# Autodesk Inventor assembly: Assembly1
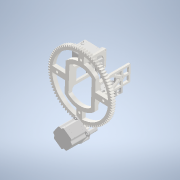
[picture p0: Inventor's stored thumbnail of the model, 180x180]
Saved by Autodesk Inventor 2020 (Build 240168000, 168)
## iProperties
Created: 2019-04-12
Part Number: Assembly1
Document SubType Name: Assembly
Designer: Connor
Author: Connor
## Documents named in this file (7)
- C:\Users\Connor\Desktop\Sentinel CAD\MainAssembly.iam
- C:\Users\Connor\Desktop\Sentinel CAD\MainAssembly\Design Accelerator\GearAssembly.iam
- C:\Users\Connor\Desktop\Sentinel CAD\HoseMount.ipt
- C:\Users\Connor\Desktop\Sentinel CAD\PK266M-01A.ipt
- C:\Users\Connor\Desktop\Sentinel CAD\TopMotorMount.ipt
- C:\Users\Connor\Desktop\Sentinel CAD\NozzleAdapter.ipt
- C:\Users\Connor\Desktop\Sentinel CAD\CameraFilterPlate.ipt
## Components (7 placed, 6 different names)
1. Spur Gears:1 [sub-assembly] — Mate:1, Mate:3, Mate:4, Flush:1, Mate:7
2. PK266M-01A:1 — Mate:1, Mate:3, Mate:4, Mate:5, Mate:6, Angle:1
3. HoseMount:1 — Mate:5, Mate:6, Angle:1, Mate:11, Mate:12, Mate:13, Mate:14, Mate:15, Mate:16
4. TopMotorMount:1 — Flush:1, Mate:7, Mate:8, Mate:9, Mate:10
5. PK266M-01A:2 — Mate:8, Mate:9, Mate:10
6. NozzleAdapter:1 — Mate:11, Mate:12, Mate:13
7. CameraFilterPlate:1 — Mate:14, Mate:15, Mate:16
## Relationships (17: Mate 15, Angle 1, Flush 1)
- Mate:1: Spur Gears:1 ↔ PK266M-01A:1
- Mate:3: Spur Gears:1 ↔ PK266M-01A:1
- Mate:4: Spur Gears:1 ↔ PK266M-01A:1
- Mate:5: PK266M-01A:1 ↔ HoseMount:1
- Mate:6: PK266M-01A:1 ↔ HoseMount:1
- Angle:1 (180 deg): PK266M-01A:1 ↔ HoseMount:1
- Flush:1 (-8.5344 mm): Spur Gears:1 ↔ TopMotorMount:1
- Mate:7: Spur Gears:1 ↔ TopMotorMount:1
- Mate:8: TopMotorMount:1 ↔ PK266M-01A:2
- Mate:9: TopMotorMount:1 ↔ PK266M-01A:2
- Mate:10: TopMotorMount:1 ↔ PK266M-01A:2
- Mate:11: HoseMount:1 ↔ NozzleAdapter:1
- Mate:12: HoseMount:1 ↔ NozzleAdapter:1
- Mate:13: HoseMount:1 ↔ NozzleAdapter:1
- Mate:14: HoseMount:1 ↔ CameraFilterPlate:1
- Mate:15: HoseMount:1 ↔ CameraFilterPlate:1
- Mate:16: HoseMount:1 ↔ CameraFilterPlate:1
